# Autodesk Inventor assembly: Máquina boca de pescado básica
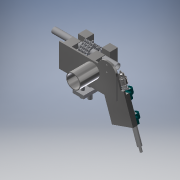
[picture p0: Inventor's stored thumbnail of the model, 180x180]
Saved by Autodesk Inventor 2018 (Build 220112000, 112)
## iProperties
Created: 2021-07-05
Part Number: Máquina boca de pescado básica
Material: Genérico
Document SubType Name: Assembly
Designer: GABRIEL
Author: GABRIEL
## Documents named in this file (19)
- C:\Users\GABRIEL\Documents\Gabriel\UNAL\SEMESTRE XI\Automatización de PM\Proyecto\Maquina de boca de pescado\Máquina boca de pescado básica.iam
- C:\Users\GABRIEL\Documents\Gabriel\Modelados\Placa1.ipt
- C:\Users\GABRIEL\Documents\Gabriel\UNAL\SEMESTRE XI\Automatización de PM\Proyecto\Maquina de boca de pescado\Base.ipt
- C:\Users\GABRIEL\Documents\Gabriel\UNAL\SEMESTRE XI\Automatización de PM\Proyecto\Maquina de boca de pescado\Posicionador.ipt
- C:\Users\GABRIEL\Documents\Gabriel\UNAL\SEMESTRE XI\Automatización de PM\Proyecto\Maquina de boca de pescado\pie.ipt
- C:\Users\GABRIEL\Documents\Gabriel\UNAL\SEMESTRE XI\Automatización de PM\Proyecto\Maquina de boca de pescado\Rodamiento.iam
- C:\Users\GABRIEL\Documents\Gabriel\UNAL\SEMESTRE XI\Automatización de PM\Proyecto\Maquina de boca de pescado\Soporte_rods.ipt
- C:\Users\GABRIEL\Documents\Gabriel\UNAL\SEMESTRE XI\Automatización de PM\Proyecto\Maquina de boca de pescado\eje.ipt
- C:\Users\GABRIEL\Documents\Gabriel\UNAL\SEMESTRE XI\Automatización de PM\Proyecto\Maquina de boca de pescado\spindle.ipt
- C:\Users\GABRIEL\Documents\Gabriel\UNAL\SEMESTRE XI\Automatización de PM\Proyecto\Maquina de boca de pescado\anclaje.ipt
- C:\Users\GABRIEL\Documents\Gabriel\UNAL\SEMESTRE XI\Automatización de PM\Proyecto\Maquina de boca de pescado\ancla.ipt
- C:\Users\GABRIEL\Documents\Gabriel\UNAL\SEMESTRE XI\Automatización de PM\Proyecto\Maquina de boca de pescado\ancla_tornillo.ipt
- C:\Users\GABRIEL\Documents\Gabriel\UNAL\SEMESTRE XI\Automatización de PM\Proyecto\Maquina de boca de pescado\sujetador.ipt
- C:\Users\GABRIEL\Documents\Gabriel\UNAL\SEMESTRE XI\Automatización de PM\Proyecto\Maquina de boca de pescado\din_912-m20x1_5-200-10_9.ipt
- C:\Users\GABRIEL\Documents\Gabriel\UNAL\SEMESTRE XI\Automatización de PM\Proyecto\Maquina de boca de pescado\encaje.ipt
- C:\Users\GABRIEL\Documents\Gabriel\UNAL\SEMESTRE XI\Automatización de PM\Proyecto\Maquina de boca de pescado\22200-0580308315.ipt
- C:\Users\GABRIEL\Documents\Gabriel\UNAL\SEMESTRE XI\Automatización de PM\Proyecto\Maquina de boca de pescado\motor_cml-30.ipt
- C:\Users\GABRIEL\Documents\Gabriel\UNAL\SEMESTRE XI\Automatización de PM\Proyecto\Maquina de boca de pescado\Tubo_ensayo.ipt
- C:\Users\GABRIEL\Documents\Gabriel\UNAL\SEMESTRE XI\Automatización de PM\Proyecto\Maquina de boca de pescado\Varilla_suj.ipt
## Components (34 placed, 18 different names)
1. Base:1 — Coincidencia:1, Nivelación:1, Nivelación:2, Coincidencia:2, Nivelación:3, Coincidencia:6, Nivelación:4, Nivelación:5, Coincidencia:11, Coincidencia:12, Ángulo:1, Coincidencia:15, Nivelación:12, Coincidencia:56
2. Soporte:1 — Coincidencia:1, Nivelación:1, Nivelación:2, Coincidencia:3, Coincidencia:16
3. Soporte:2 — Coincidencia:2, Nivelación:3, Coincidencia:3, Coincidencia:7, Tangente:1, Tangente:2
4. pie:1 — Coincidencia:6, Nivelación:4, Nivelación:5, Coincidencia:7
5. Posicionador:1 — Coincidencia:8, Nivelación:6, Nivelación:7, Coincidencia:11, Coincidencia:12, Ángulo:1, Coincidencia:57, Coincidencia:59
6. Rodamiento:1 [sub-assembly] — Coincidencia:9, Nivelación:8, Nivelación:9, Insertar:1
7. Rodamiento:2 [sub-assembly] — Coincidencia:10, Nivelación:10, Nivelación:11
8. Soporte_rods:1 — Coincidencia:8, Nivelación:6, Nivelación:7, Coincidencia:9, Nivelación:8, Nivelación:9, Coincidencia:10, Nivelación:10, Nivelación:11
9. eje:1 — Insertar:1, Coincidencia:13, Coincidencia:14, Rotación:1
10. spindle:1 — Coincidencia:13, Coincidencia:14, Rotación:1
11. anclaje:1 — Coincidencia:15, Nivelación:12, Coincidencia:16, Coincidencia:17, Coincidencia:18, Coincidencia:19, Coincidencia:20, Coincidencia:21, Coincidencia:22, Ángulo:2, Coincidencia:26, Ángulo:3, Coincidencia:61
12. ancla:1 — Coincidencia:17, Coincidencia:18, Coincidencia:23, Coincidencia:25
13. ancla:2 — Coincidencia:19, Coincidencia:20, Coincidencia:24
14. ancla_tornillo:1 — Coincidencia:21, Coincidencia:22, Coincidencia:60
15. sujetador:1 — Insertar:2, Insertar:3, Coincidencia:25, Nivelación:13
16. din_912-m20x1_5-200-10_9:1 — Insertar:3, Coincidencia:24, Insertar:5
17. din_912-m20x1_5-200-10_9:2 — Insertar:2, Coincidencia:23, Insertar:4
18. encaje:1 — Insertar:4, Ángulo:2, Coincidencia:26, Coincidencia:27, Coincidencia:30, Coincidencia:31, Coincidencia:49, Coincidencia:52, Coincidencia:54
19. encaje:2 — Insertar:5, Ángulo:3, Coincidencia:36, Coincidencia:50, Coincidencia:53
20. 22200-0580308315:1 — Coincidencia:27, Coincidencia:28, Coincidencia:29, Coincidencia:30, Coincidencia:31, Coincidencia:51
21. 22200-0580308315:2 — Coincidencia:28, Coincidencia:29, Coincidencia:32, Coincidencia:33, Tangente:8, Tangente:9
22. 22200-0580308315:3 — Coincidencia:32, Coincidencia:33, Coincidencia:34, Coincidencia:35, Tangente:10
23. 22200-0580308315:5 — Coincidencia:34, Coincidencia:35, Coincidencia:36
24. 22200-0580308315:6 — Coincidencia:52, Coincidencia:54, Coincidencia:55
25. 22200-0580308315:7 — Tangente:4, Tangente:5
26. 22200-0580308315:8 — Tangente:3
27. 22200-0580308315:9 — Coincidencia:53
28. 22200-0580308315:10 — Coincidencia:49, Coincidencia:51, Coincidencia:55
29. 22200-0580308315:11 — Tangente:6
30. 22200-0580308315:12 — Tangente:7, Tangente:11
31. 22200-0580308315:13 — Coincidencia:50
32. motor_cml-30:1 — Coincidencia:56, Coincidencia:57, Coincidencia:59
33. Tubo_ensayo:1 — Tangente:1, Tangente:2, Tangente:3, Tangente:4, Tangente:5, Tangente:6, Tangente:7, Tangente:8, Tangente:9, Tangente:10, Tangente:11
34. Varilla_suj:1 — Coincidencia:60, Coincidencia:61, Nivelación:13
## Relationships (91: Mate 58, Flush 13, Tangent 11, Insert 5, Angle 3, RelateRotation 1)
- Coincidencia:1 [Mate]: Base:1 ↔ Soporte:1
- Nivelación:1 [Flush] (10 mm): Base:1 ↔ Soporte:1
- Nivelación:2 [Flush] (-10 mm): Base:1 ↔ Soporte:1
- Coincidencia:2 [Mate]: Base:1 ↔ Soporte:2
- Nivelación:3 [Flush] (10 mm): Base:1 ↔ Soporte:2
- Coincidencia:3 [Mate] (100 mm): Soporte:1 ↔ Soporte:2
- Coincidencia:6 [Mate]: Base:1 ↔ pie:1
- Nivelación:4 [Flush]: Base:1 ↔ pie:1
- Nivelación:5 [Flush] (10 mm): Base:1 ↔ pie:1
- Coincidencia:7 [Mate]: Soporte:2 ↔ pie:1
- Coincidencia:8 [Mate]: Posicionador:1 ↔ Soporte_rods:1
- Nivelación:6 [Flush]: Posicionador:1 ↔ Soporte_rods:1
- Nivelación:7 [Flush]: Posicionador:1 ↔ Soporte_rods:1
- Coincidencia:9 [Mate]: Rodamiento:1 ↔ Soporte_rods:1
- Nivelación:8 [Flush]: Rodamiento:1 ↔ Soporte_rods:1
- Nivelación:9 [Flush]: Rodamiento:1 ↔ Soporte_rods:1
- Coincidencia:10 [Mate]: Rodamiento:2 ↔ Soporte_rods:1
- Nivelación:10 [Flush]: Rodamiento:2 ↔ Soporte_rods:1
- Nivelación:11 [Flush]: Rodamiento:2 ↔ Soporte_rods:1
- Coincidencia:11 [Mate]: Base:1 ↔ Posicionador:1
- Coincidencia:12 [Mate]: Base:1 ↔ Posicionador:1
- Ángulo:1 [Angle] (0 deg): Base:1 ↔ Posicionador:1
- Insertar:1 (-20 mm): Rodamiento:1 ↔ eje:1
- Coincidencia:13 [Mate]: eje:1 ↔ spindle:1
- Coincidencia:14 [Mate]: eje:1 ↔ spindle:1
- Rotación:1 [RelateRotation] (1 ul): eje:1 ↔ spindle:1
- Coincidencia:15 [Mate]: Base:1 ↔ anclaje:1
- Nivelación:12 [Flush] (10 mm): Base:1 ↔ anclaje:1
- Coincidencia:16 [Mate] (10 mm): Soporte:1 ↔ anclaje:1
- Coincidencia:17 [Mate]: anclaje:1 ↔ ancla:1
- Coincidencia:18 [Mate]: anclaje:1 ↔ ancla:1
- Coincidencia:19 [Mate]: anclaje:1 ↔ ancla:2
- Coincidencia:20 [Mate]: anclaje:1 ↔ ancla:2
- Coincidencia:21 [Mate]: anclaje:1 ↔ ancla_tornillo:1
- Coincidencia:22 [Mate]: anclaje:1 ↔ ancla_tornillo:1
- Insertar:2: sujetador:1 ↔ din_912-m20x1_5-200-10_9:2
- Insertar:3: sujetador:1 ↔ din_912-m20x1_5-200-10_9:1
- Coincidencia:23 [Mate]: ancla:1 ↔ din_912-m20x1_5-200-10_9:2
- Coincidencia:24 [Mate]: ancla:2 ↔ din_912-m20x1_5-200-10_9:1
- Coincidencia:25 [Mate]: ancla:1 ↔ sujetador:1
- Insertar:4 (-10 mm): din_912-m20x1_5-200-10_9:2 ↔ encaje:1
- Ángulo:2 [Angle] (0 deg): anclaje:1 ↔ encaje:1
- Coincidencia:26 [Mate]: anclaje:1 ↔ encaje:1
- Insertar:5 (-15 mm): din_912-m20x1_5-200-10_9:1 ↔ encaje:2
- Ángulo:3 [Angle] (0 deg): anclaje:1 ↔ encaje:2
- Coincidencia:27 [Mate]: encaje:1 ↔ 22200-0580308315:1
- Coincidencia:28 [Mate]: 22200-0580308315:1 ↔ 22200-0580308315:2
- Coincidencia:29 [Mate]: 22200-0580308315:1 ↔ 22200-0580308315:2
- Coincidencia:30 [Mate]: encaje:1 ↔ 22200-0580308315:1
- Coincidencia:31 [Mate]: encaje:1 ↔ 22200-0580308315:1
- Coincidencia:32 [Mate]: 22200-0580308315:2 ↔ 22200-0580308315:3
- Coincidencia:33 [Mate]: 22200-0580308315:2 ↔ 22200-0580308315:3
- Coincidencia:34 [Mate]: 22200-0580308315:3 ↔ 22200-0580308315:5
- Coincidencia:35 [Mate]: 22200-0580308315:3 ↔ 22200-0580308315:5
- Coincidencia:36 [Mate]: encaje:2 ↔ 22200-0580308315:5
- [Mate]: 22200-0580308315:6 ↔ 22200-0580308315:7
- [Mate]: 22200-0580308315:6 ↔ 22200-0580308315:7
- [Mate]: 22200-0580308315:7 ↔ 22200-0580308315:8
- [Mate]: 22200-0580308315:7 ↔ 22200-0580308315:8
- [Mate]: 22200-0580308315:8 ↔ 22200-0580308315:9
- [Mate]: 22200-0580308315:8 ↔ 22200-0580308315:9
- [Mate]: 22200-0580308315:10 ↔ 22200-0580308315:11
- [Mate]: 22200-0580308315:10 ↔ 22200-0580308315:11
- [Mate]: 22200-0580308315:11 ↔ 22200-0580308315:12
- [Mate]: 22200-0580308315:11 ↔ 22200-0580308315:12
- [Mate]: 22200-0580308315:12 ↔ 22200-0580308315:13
- [Mate]: 22200-0580308315:12 ↔ 22200-0580308315:13
- Coincidencia:49 [Mate]: encaje:1 ↔ 22200-0580308315:10
- Coincidencia:50 [Mate]: encaje:2 ↔ 22200-0580308315:13
- Coincidencia:51 [Mate]: 22200-0580308315:1 ↔ 22200-0580308315:10
- Coincidencia:52 [Mate]: encaje:1 ↔ 22200-0580308315:6
- Coincidencia:53 [Mate]: encaje:2 ↔ 22200-0580308315:9
- Coincidencia:54 [Mate]: encaje:1 ↔ 22200-0580308315:6
- Coincidencia:55 [Mate]: 22200-0580308315:6 ↔ 22200-0580308315:10
- Coincidencia:56 [Mate]: Base:1 ↔ motor_cml-30:1
- Coincidencia:57 [Mate]: Posicionador:1 ↔ motor_cml-30:1
- Coincidencia:59 [Mate]: Posicionador:1 ↔ motor_cml-30:1
- Tangente:1: Soporte:2 ↔ Tubo_ensayo:1
- Tangente:2: Soporte:2 ↔ Tubo_ensayo:1
- Tangente:3: 22200-0580308315:8 ↔ Tubo_ensayo:1
- Tangente:4: 22200-0580308315:7 ↔ Tubo_ensayo:1
- Tangente:5: 22200-0580308315:7 ↔ Tubo_ensayo:1
- Tangente:6: 22200-0580308315:11 ↔ Tubo_ensayo:1
- Tangente:7: 22200-0580308315:12 ↔ Tubo_ensayo:1
- Tangente:8: 22200-0580308315:2 ↔ Tubo_ensayo:1
- Tangente:9: 22200-0580308315:2 ↔ Tubo_ensayo:1
- Tangente:10: 22200-0580308315:3 ↔ Tubo_ensayo:1
- Tangente:11: 22200-0580308315:12 ↔ Tubo_ensayo:1
- Coincidencia:60 [Mate]: ancla_tornillo:1 ↔ Varilla_suj:1
- Coincidencia:61 [Mate]: anclaje:1 ↔ Varilla_suj:1
- Nivelación:13 [Flush] (-50 mm): sujetador:1 ↔ Varilla_suj:1
## Named parameters: d77_d73 = 0 mm, d78_d74 = 0 mm, d79_d75 = 0 mm, d80_d64 = 0 mm, d81_d65 = 0 mm, d82_d72 = 0 mm, d83_d73 = 0 mm, d84_d74 = 0 mm, d85_d75 = 0 mm, d86_d64 = 0 mm, d87_d65 = 0 mm, d88_d72 = 0 mm
